# Autodesk Inventor assembly: DONE
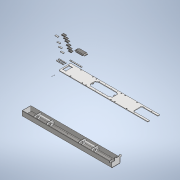
[picture p0: Inventor's stored thumbnail of the model, 180x180]
Saved by Autodesk Inventor 2020 (Build 240168000, 168)
## iProperties
Created: 2022-10-21
Part Number: DONE
Document SubType Name: Assembly
Designer: lura02001
Author: lura02001
## Documents named in this file (14)
- H:\sliperlåda\DONE.iam
- H:\sliperlåda\SlipersLåda 211018001.ipt
- H:\sliperlåda\SlipersLåda 211018004.ipt
- H:\sliperlåda\SlipersLåda 211018004-1.ipt
- H:\sliperlåda\SlipersLåda 211018007.ipt
- H:\sliperlåda\SlipersLåda 211018005.ipt
- H:\sliperlåda\SlipersLåda 211018006.ipt
- H:\sliperlåda\SlipersLåda 211018008.ipt
- H:\sliperlåda\SlipersLåda 211018011.ipt
- H:\sliperlåda\SlipersLåda 211018010.ipt
- H:\sliperlåda\SlipersLåda 211018012.ipt
- H:\sliperlåda\SlipersLåda 211018009.ipt
- H:\sliperlåda\SlipersLåda 211018002.ipt
- H:\Ritningsläsning\öv2pt2.ipt
## Components (28 placed, 13 different names)
1. SlipersLåda 211018001:1 — Mate:3, Flush:2, Flush:3, Mate:4, Mate:5, Mate:6, Mate:7, Mate:9, Mate:10, Mate:12, Mate:13, Mate:15, Mate:16
2. SlipersLåda 211018004:1 — Mate:12, Mate:13, Mate:14, Mate:20, Mate:21
3. SlipersLåda 211018004:2 — Mate:15, Mate:16, Mate:17, Mate:18, Flush:4, Mate:19
4. SlipersLåda 211018004-1:2 — Mate:9, Mate:10, Mate:11, Mate:22, Flush:5, Flush:6
5. SlipersLåda 211018007:1
6. SlipersLåda 211018007:2
7. SlipersLåda 211018005:1 — Mate:19, Mate:20, Mate:21
8. SlipersLåda 211018005:2 — Mate:18, Flush:4
9. SlipersLåda 211018005:3 — Mate:22, Mate:23, Flush:5
10. SlipersLåda 211018005:4 — Mate:24, Flush:6
11. SlipersLåda 211018006:1
12. SlipersLåda 211018008:1
13. SlipersLåda 211018008:2
14. SlipersLåda 211018008:3
15. SlipersLåda 211018008:4
16. SlipersLåda 211018011:1
17. SlipersLåda 211018011:2
18. SlipersLåda 211018011:3
19. SlipersLåda 211018011:4
20. SlipersLåda 211018011:5
21. SlipersLåda 211018011:6
22. SlipersLåda 211018010:1
23. SlipersLåda 211018010:2
24. SlipersLåda 211018012:1
25. SlipersLåda 211018009:1
26. SlipersLåda 211018002:1 — Mate:3, Flush:2, Mate:14, Mate:17
27. öv2pt2:1 — Flush:3, Mate:4, Mate:5, Mate:8, Mate:11
28. SlipersLåda 211018004:3 — Mate:6, Mate:7, Mate:8, Mate:23, Mate:24
## Relationships (27: Mate 22, Flush 5)
- Mate:3: SlipersLåda 211018001:1 ↔ SlipersLåda 211018002:1
- Flush:2: SlipersLåda 211018001:1 ↔ SlipersLåda 211018002:1
- Flush:3: SlipersLåda 211018001:1 ↔ öv2pt2:1
- Mate:4 (1 mm): SlipersLåda 211018001:1 ↔ öv2pt2:1
- Mate:5 (1 mm): SlipersLåda 211018001:1 ↔ öv2pt2:1
- Mate:6: SlipersLåda 211018001:1 ↔ SlipersLåda 211018004:3
- Mate:7: SlipersLåda 211018001:1 ↔ SlipersLåda 211018004:3
- Mate:8 (710 mm): öv2pt2:1 ↔ SlipersLåda 211018004:3
- Mate:9: SlipersLåda 211018001:1 ↔ SlipersLåda 211018004-1:2
- Mate:10: SlipersLåda 211018001:1 ↔ SlipersLåda 211018004-1:2
- Mate:11 (1130 mm): SlipersLåda 211018004-1:2 ↔ öv2pt2:1
- Mate:12: SlipersLåda 211018001:1 ↔ SlipersLåda 211018004:1
- Mate:13: SlipersLåda 211018001:1 ↔ SlipersLåda 211018004:1
- Mate:14 (345 mm): SlipersLåda 211018004:1 ↔ SlipersLåda 211018002:1
- Mate:15: SlipersLåda 211018001:1 ↔ SlipersLåda 211018004:2
- Mate:16: SlipersLåda 211018001:1 ↔ SlipersLåda 211018004:2
- Mate:17 (765 mm): SlipersLåda 211018004:2 ↔ SlipersLåda 211018002:1
- Mate:18: SlipersLåda 211018004:2 ↔ SlipersLåda 211018005:2
- Flush:4 (-40 mm): SlipersLåda 211018004:2 ↔ SlipersLåda 211018005:2
- Mate:19: SlipersLåda 211018004:2 ↔ SlipersLåda 211018005:1
- Mate:20 (40 mm): SlipersLåda 211018004:1 ↔ SlipersLåda 211018005:1
- Mate:21: SlipersLåda 211018004:1 ↔ SlipersLåda 211018005:1
- Mate:22: SlipersLåda 211018004-1:2 ↔ SlipersLåda 211018005:3
- Mate:23: SlipersLåda 211018005:3 ↔ SlipersLåda 211018004:3
- Flush:5 (-40 mm): SlipersLåda 211018004-1:2 ↔ SlipersLåda 211018005:3
- Mate:24: SlipersLåda 211018005:4 ↔ SlipersLåda 211018004:3
- Flush:6 (-40 mm): SlipersLåda 211018004-1:2 ↔ SlipersLåda 211018005:4
